# Autodesk Inventor assembly: Ensamble
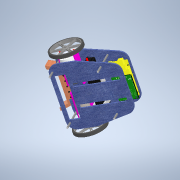
[picture p0: Inventor's stored thumbnail of the model, 180x180]
Saved by Autodesk Inventor 2020 (Build 240168000, 168)
## iProperties
Created: 2020-11-22
Part Number: Ensamble
Document SubType Name: Assembly
Designer: michelin
Author: michelin
## Documents named in this file (16)
- C:\Users\michelin\Desktop\Segundo semestre\Fundamentos de robótica\Tarea5\Ensamble.iam
- C:\Users\michelin\Desktop\Segundo semestre\Fundamentos de robótica\Tarea5\37d-gearmotor-50-70-encoder.ipt
- C:\Users\michelin\Desktop\Segundo semestre\Fundamentos de robótica\Tarea5\Base.ipt
- C:\Users\michelin\Desktop\Segundo semestre\Fundamentos de robótica\Tarea5\tapa.ipt
- C:\Users\michelin\Desktop\Segundo semestre\Fundamentos de robótica\Tarea5\Porta pilas.ipt
- C:\Users\michelin\Desktop\Segundo semestre\Fundamentos de robótica\Tarea5\Bateria.ipt
- C:\Users\michelin\Desktop\Segundo semestre\Fundamentos de robótica\Tarea5\ArduinoMega_STEP_AP203.ipt
- C:\Users\michelin\Desktop\Segundo semestre\Fundamentos de robótica\Tarea5\pololu-wheel-90x10mm-black.ipt
- C:\Users\michelin\Desktop\Segundo semestre\Fundamentos de robótica\Tarea5\pololu-dual-vnh5019-motor-driver-shield.ipt
- C:\Users\michelin\Desktop\Segundo semestre\Fundamentos de robótica\Tarea5\Rueda trasera.ipt
- C:\Users\michelin\Desktop\Segundo semestre\Fundamentos de robótica\Tarea5\Soporte motor.ipt
- C:\Users\michelin\Desktop\Segundo semestre\Fundamentos de robótica\Tarea5\Tapa motor.ipt
- C:\Users\michelin\Desktop\Segundo semestre\Fundamentos de robótica\Tarea5\tornillo M3 corto.ipt
- C:\Users\michelin\Desktop\Segundo semestre\Fundamentos de robótica\Tarea5\pololu-universal-aluminum-mounting-hub-for-6mm-shaft-4-40-holes.ipt
- C:\Users\michelin\Desktop\Segundo semestre\Fundamentos de robótica\Tarea5\tornillo M5 largo.ipt
- C:\Users\michelin\Desktop\Segundo semestre\Fundamentos de robótica\Tarea5\Pala.ipt
## Components (49 placed, 15 different names)
1. 37d-gearmotor-50-70-encoder:1 — Flush:3, Mate:17, Mate:24, Mate:25
2. 37d-gearmotor-50-70-encoder:2 — Flush:4, Mate:28, Mate:35
3. Base:1 — Mate:4, Mate:5, Mate:6, Mate:7, Mate:8, Mate:9, Mate:10, Mate:11, Mate:12, Mate:14, Mate:15, Mate:16, Mate:21, Mate:22, Mate:23, Rotational:6, Rotational:7, Rotational:8, Rotational:9, Mate:39, Mate:40, Mate:41, Rigid:1, Rotational:15, Rigid:2, Rotational:16, Rotational:17, Rotational:18, Rotational:21, Rotational:22, Rotational:23, Rotational:24, Rotational:25, Rotational:26, Rotational:27, Rotational:28, Rotational:29, Rotational:30
4. Porta pilas:1 — Mate:1, Mate:2, Mate:3, Mate:4, Mate:5, Mate:6
5. Bateria:1 — Mate:1, Mate:2, Mate:3
6. ArduinoMega_STEP_AP203:1 — Mate:7, Mate:8, Mate:9, Mate:13, Flush:1, Flush:2
7. pololu-wheel-90x10mm-black:1 — Mate:34, Mate:35
8. pololu-wheel-90x10mm-black:2 — Mate:26, Mate:27
9. Rueda trasera:1 — Mate:10, Mate:11, Mate:12, Rotational:19, Rotational:20
10. pololu-dual-vnh5019-motor-driver-shield:1 — Mate:13, Flush:1, Flush:2
11. Soporte motor:1 — Mate:14, Mate:15, Mate:16, Flush:3, Mate:17, Mate:18, Mate:19, Mate:20
12. Soporte motor:2 — Mate:21, Mate:22, Mate:23, Flush:4, Mate:28, Mate:29, Mate:30, Mate:31
13. Tapa motor:1 — Mate:18, Mate:19, Mate:20, Rotational:1, Rotational:2
14. tornillo M3 corto:1 — Rotational:1
15. tornillo M3 corto:2 — Rotational:2
16. tornillo M3 corto:3 — Rotational:3
17. pololu-universal-aluminum-mounting-hub-for-6mm-shaft-4-40-holes:1 — Mate:24, Mate:25, Mate:26, Mate:27
18. Tapa motor:2 — Mate:29, Mate:30, Mate:31, Rotational:3, Rotational:4, Mate:32, Mate:33
19. tornillo M3 corto:4 — Rotational:4
20. pololu-universal-aluminum-mounting-hub-for-6mm-shaft-4-40-holes:2 — Mate:32, Mate:33, Mate:34
21. tornillo M5 largo:2 — Rotational:7, Mate:36, Mate:38
22. tornillo M5 largo:3 — Rotational:8
23. tornillo M5 largo:4 — Rotational:6, Mate:37
24. tapa:1 — Mate:36, Mate:37, Mate:38
25. tornillo M5 largo:5 — Rotational:9
26. Pala:1 — Mate:39, Mate:40, Mate:41, Rotational:10, Rotational:11, Rotational:12, Rotational:13, Rotational:14
27. tornillo M3 corto:5 — Rotational:12
28. tornillo M3 corto:6 — Rotational:10
29. tornillo M3 corto:7 — Rotational:13
30. tornillo M3 corto:8 — Rotational:11
31. tornillo M3 corto:10 — Rotational:14
32. tornillo M3 corto:12 — Rotational:16
33. tornillo M3 corto:13 — Rotational:15
34. tornillo M3 corto:14 — Rigid:1
35. tornillo M3 corto:15 — Rigid:2
36. tornillo M3 corto:16 — Rotational:17
37. tornillo M3 corto:17 — Rotational:22
38. tornillo M3 corto:18 — Rotational:18
39. tornillo M3 corto:19 — Rotational:20
40. tornillo M3 corto:20 — Rotational:23
41. tornillo M3 corto:21 — Rotational:19
42. tornillo M3 corto:22 — Rotational:21
43. tornillo M3 corto:23 — Rotational:24
44. tornillo M3 corto:24 — Rotational:28
45. tornillo M3 corto:25 — Rotational:25
46. tornillo M3 corto:26 — Rotational:26
47. tornillo M3 corto:27 — Rotational:29
48. tornillo M3 corto:28 — Rotational:27
49. tornillo M3 corto:29 — Rotational:30
## Relationships (76: Mate 41, RevoluteJoint 29, Flush 4, WeldJoint 2)
- Mate:1: Porta pilas:1 ↔ Bateria:1
- Mate:2: Porta pilas:1 ↔ Bateria:1
- Mate:3: Porta pilas:1 ↔ Bateria:1
- Mate:4: Base:1 ↔ Porta pilas:1
- Mate:5: Base:1 ↔ Porta pilas:1
- Mate:6: Base:1 ↔ Porta pilas:1
- Mate:7: Base:1 ↔ ArduinoMega_STEP_AP203:1
- Mate:8: Base:1 ↔ ArduinoMega_STEP_AP203:1
- Mate:9: Base:1 ↔ ArduinoMega_STEP_AP203:1
- Mate:10: Base:1 ↔ Rueda trasera:1
- Mate:11: Base:1 ↔ Rueda trasera:1
- Mate:12: Base:1 ↔ Rueda trasera:1
- Mate:13: ArduinoMega_STEP_AP203:1 ↔ pololu-dual-vnh5019-motor-driver-shield:1
- Flush:1: ArduinoMega_STEP_AP203:1 ↔ pololu-dual-vnh5019-motor-driver-shield:1
- Flush:2: ArduinoMega_STEP_AP203:1 ↔ pololu-dual-vnh5019-motor-driver-shield:1
- Mate:14: Base:1 ↔ Soporte motor:1
- Mate:15: Base:1 ↔ Soporte motor:1
- Mate:16: Base:1 ↔ Soporte motor:1
- Flush:3: 37d-gearmotor-50-70-encoder:1 ↔ Soporte motor:1
- Mate:17: 37d-gearmotor-50-70-encoder:1 ↔ Soporte motor:1
- Mate:18: Soporte motor:1 ↔ Tapa motor:1
- Mate:19: Soporte motor:1 ↔ Tapa motor:1
- Mate:20: Soporte motor:1 ↔ Tapa motor:1
- Mate:21: Base:1 ↔ Soporte motor:2
- Mate:22: Base:1 ↔ Soporte motor:2
- Mate:23: Base:1 ↔ Soporte motor:2
- Rotational:1 [RevoluteJoint]: Tapa motor:1 ↔ tornillo M3 corto:1
- Rotational:2 [RevoluteJoint]: Tapa motor:1 ↔ tornillo M3 corto:2
- Mate:24: 37d-gearmotor-50-70-encoder:1 ↔ pololu-universal-aluminum-mounting-hub-for-6mm-shaft-4-40-holes:1
- Mate:25: 37d-gearmotor-50-70-encoder:1 ↔ pololu-universal-aluminum-mounting-hub-for-6mm-shaft-4-40-holes:1
- Mate:26: pololu-wheel-90x10mm-black:2 ↔ pololu-universal-aluminum-mounting-hub-for-6mm-shaft-4-40-holes:1
- Mate:27: pololu-wheel-90x10mm-black:2 ↔ pololu-universal-aluminum-mounting-hub-for-6mm-shaft-4-40-holes:1
- Flush:4: 37d-gearmotor-50-70-encoder:2 ↔ Soporte motor:2
- Mate:28: 37d-gearmotor-50-70-encoder:2 ↔ Soporte motor:2
- Mate:29: Soporte motor:2 ↔ Tapa motor:2
- Mate:30: Soporte motor:2 ↔ Tapa motor:2
- Mate:31: Soporte motor:2 ↔ Tapa motor:2
- Rotational:3 [RevoluteJoint]: tornillo M3 corto:3 ↔ Tapa motor:2
- Rotational:4 [RevoluteJoint]: Tapa motor:2 ↔ tornillo M3 corto:4
- Mate:32: Tapa motor:2 ↔ pololu-universal-aluminum-mounting-hub-for-6mm-shaft-4-40-holes:2
- Mate:33: Tapa motor:2 ↔ pololu-universal-aluminum-mounting-hub-for-6mm-shaft-4-40-holes:2
- Mate:34: pololu-wheel-90x10mm-black:1 ↔ pololu-universal-aluminum-mounting-hub-for-6mm-shaft-4-40-holes:2
- Mate:35: 37d-gearmotor-50-70-encoder:2 ↔ pololu-wheel-90x10mm-black:1
- Rotational:6 [RevoluteJoint]: Base:1 ↔ tornillo M5 largo:4
- Rotational:7 [RevoluteJoint]: Base:1 ↔ tornillo M5 largo:2
- Mate:36: tornillo M5 largo:2 ↔ tapa:1
- Mate:37: tornillo M5 largo:4 ↔ tapa:1
- Mate:38: tornillo M5 largo:2 ↔ tapa:1
- Rotational:8 [RevoluteJoint]: Base:1 ↔ tornillo M5 largo:3
- Rotational:9 [RevoluteJoint]: Base:1 ↔ tornillo M5 largo:5
- Mate:39: Base:1 ↔ Pala:1
- Mate:40: Base:1 ↔ Pala:1
- Mate:41: Base:1 ↔ Pala:1
- Rotational:10 [RevoluteJoint]: Pala:1 ↔ tornillo M3 corto:6
- Rotational:11 [RevoluteJoint]: Pala:1 ↔ tornillo M3 corto:8
- Rotational:12 [RevoluteJoint]: Pala:1 ↔ tornillo M3 corto:5
- Rotational:13 [RevoluteJoint]: Pala:1 ↔ tornillo M3 corto:7
- Rotational:14 [RevoluteJoint]: Pala:1 ↔ tornillo M3 corto:10
- Rigid:1 [WeldJoint]: Base:1 ↔ tornillo M3 corto:14
- Rotational:15 [RevoluteJoint]: Base:1 ↔ tornillo M3 corto:13
- Rigid:2 [WeldJoint]: Base:1 ↔ tornillo M3 corto:15
- Rotational:16 [RevoluteJoint]: Base:1 ↔ tornillo M3 corto:12
- Rotational:17 [RevoluteJoint]: Base:1 ↔ tornillo M3 corto:16
- Rotational:18 [RevoluteJoint]: Base:1 ↔ tornillo M3 corto:18
- Rotational:19 [RevoluteJoint]: Rueda trasera:1 ↔ tornillo M3 corto:21
- Rotational:20 [RevoluteJoint]: Rueda trasera:1 ↔ tornillo M3 corto:19
- Rotational:21 [RevoluteJoint]: Base:1 ↔ tornillo M3 corto:22
- Rotational:22 [RevoluteJoint]: Base:1 ↔ tornillo M3 corto:17
- Rotational:23 [RevoluteJoint]: Base:1 ↔ tornillo M3 corto:20
- Rotational:24 [RevoluteJoint]: Base:1 ↔ tornillo M3 corto:23
- Rotational:25 [RevoluteJoint]: Base:1 ↔ tornillo M3 corto:25
- Rotational:26 [RevoluteJoint]: Base:1 ↔ tornillo M3 corto:26
- Rotational:27 [RevoluteJoint]: Base:1 ↔ tornillo M3 corto:28
- Rotational:28 [RevoluteJoint]: Base:1 ↔ tornillo M3 corto:24
- Rotational:29 [RevoluteJoint]: Base:1 ↔ tornillo M3 corto:27
- Rotational:30 [RevoluteJoint]: Base:1 ↔ tornillo M3 corto:29
